(part 1 of 2)
# Autodesk Inventor assembly: Waffling60-MX
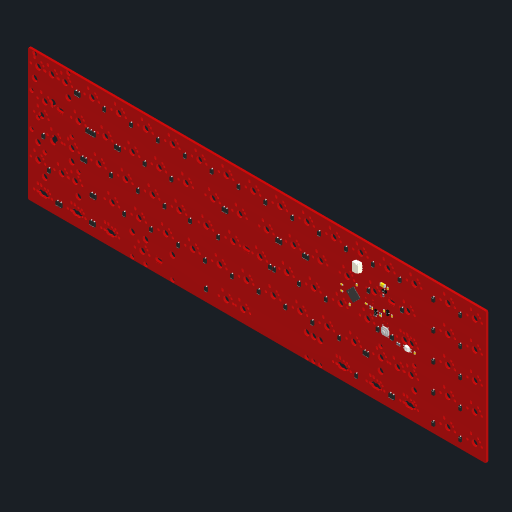
[picture p0: Inventor's stored thumbnail of the model, 512x512]
Saved by Autodesk Inventor 2024 (Build 280153000, 153)
## iProperties
Company: Open CASCADE
Created: 2024-04-27
Part Number: Waffling60-MX
Description: Open CASCADE Model
Document SubType Name: Assembly
Designer: bln15
Authority: Unknown
Sending System: Open CASCADE 7.5
Preprocessor: Open CASCADE STEP processor 7.5
Title: Open CASCADE Shape Model
Author: Author
## Documents named in this file (413)
- C:\Users\bln15\Documents\GitHub\waffling60\waffling60-XT\Waffling60-MX\Waffling60-MX.iam
- C:\Users\bln15\Documents\GitHub\waffling60\waffling60-XT\Waffling60-MX\Open CASCADE STEP translator 7.5 413.ipt
- C:\Users\bln15\Documents\GitHub\waffling60\waffling60-XT\Waffling60-MX\Open CASCADE STEP translator 7.5 414.ipt
- C:\Users\bln15\Documents\GitHub\waffling60\waffling60-XT\Waffling60-MX\Open CASCADE STEP translator 7.5 415.ipt
- C:\Users\bln15\Documents\GitHub\waffling60\waffling60-XT\Waffling60-MX\Open CASCADE STEP translator 7.5 416.ipt
- C:\Users\bln15\Documents\GitHub\waffling60\waffling60-XT\Waffling60-MX\Open CASCADE STEP translator 7.5 417.ipt
- C:\Users\bln15\Documents\GitHub\waffling60\waffling60-XT\Waffling60-MX\Open CASCADE STEP translator 7.5 418.ipt
- C:\Users\bln15\Documents\GitHub\waffling60\waffling60-XT\Waffling60-MX\Open CASCADE STEP translator 7.5 419.ipt
- C:\Users\bln15\Documents\GitHub\waffling60\waffling60-XT\Waffling60-MX\Open CASCADE STEP translator 7.5 420.ipt
- C:\Users\bln15\Documents\GitHub\waffling60\waffling60-XT\Waffling60-MX\Open CASCADE STEP translator 7.5 421.ipt
- C:\Users\bln15\Documents\GitHub\waffling60\waffling60-XT\Waffling60-MX\Open CASCADE STEP translator 7.5 422.ipt
- C:\Users\bln15\Documents\GitHub\waffling60\waffling60-XT\Waffling60-MX\Open CASCADE STEP translator 7.5 423.ipt
- C:\Users\bln15\Documents\GitHub\waffling60\waffling60-XT\Waffling60-MX\Open CASCADE STEP translator 7.5 424.ipt
- C:\Users\bln15\Documents\GitHub\waffling60\waffling60-XT\Waffling60-MX\Open CASCADE STEP translator 7.5 425.ipt
- C:\Users\bln15\Documents\GitHub\waffling60\waffling60-XT\Waffling60-MX\Open CASCADE STEP translator 7.5 426.ipt
- C:\Users\bln15\Documents\GitHub\waffling60\waffling60-XT\Waffling60-MX\Open CASCADE STEP translator 7.5 427.ipt
- C:\Users\bln15\Documents\GitHub\waffling60\waffling60-XT\Waffling60-MX\Open CASCADE STEP translator 7.5 428.ipt
- C:\Users\bln15\Documents\GitHub\waffling60\waffling60-XT\Waffling60-MX\Open CASCADE STEP translator 7.5 429.ipt
- C:\Users\bln15\Documents\GitHub\waffling60\waffling60-XT\Waffling60-MX\Open CASCADE STEP translator 7.5 430.ipt
- C:\Users\bln15\Documents\GitHub\waffling60\waffling60-XT\Waffling60-MX\Open CASCADE STEP translator 7.5 431.ipt
- C:\Users\bln15\Documents\GitHub\waffling60\waffling60-XT\Waffling60-MX\Open CASCADE STEP translator 7.5 432.ipt
- C:\Users\bln15\Documents\GitHub\waffling60\waffling60-XT\Waffling60-MX\Open CASCADE STEP translator 7.5 433.ipt
- C:\Users\bln15\Documents\GitHub\waffling60\waffling60-XT\Waffling60-MX\Open CASCADE STEP translator 7.5 434.ipt
- C:\Users\bln15\Documents\GitHub\waffling60\waffling60-XT\Waffling60-MX\Open CASCADE STEP translator 7.5 435.ipt
- C:\Users\bln15\Documents\GitHub\waffling60\waffling60-XT\Waffling60-MX\Open CASCADE STEP translator 7.5 436.ipt
- C:\Users\bln15\Documents\GitHub\waffling60\waffling60-XT\Waffling60-MX\Open CASCADE STEP translator 7.5 437.ipt
- C:\Users\bln15\Documents\GitHub\waffling60\waffling60-XT\Waffling60-MX\Open CASCADE STEP translator 7.5 438.ipt
- C:\Users\bln15\Documents\GitHub\waffling60\waffling60-XT\Waffling60-MX\Open CASCADE STEP translator 7.5 439.ipt
- C:\Users\bln15\Documents\GitHub\waffling60\waffling60-XT\Waffling60-MX\Open CASCADE STEP translator 7.5 440.ipt
- C:\Users\bln15\Documents\GitHub\waffling60\waffling60-XT\Waffling60-MX\Open CASCADE STEP translator 7.5 441.ipt
- C:\Users\bln15\Documents\GitHub\waffling60\waffling60-XT\Waffling60-MX\Open CASCADE STEP translator 7.5 442.ipt
- C:\Users\bln15\Documents\GitHub\waffling60\waffling60-XT\Waffling60-MX\Open CASCADE STEP translator 7.5 443.ipt
- C:\Users\bln15\Documents\GitHub\waffling60\waffling60-XT\Waffling60-MX\Open CASCADE STEP translator 7.5 444.ipt
- C:\Users\bln15\Documents\GitHub\waffling60\waffling60-XT\Waffling60-MX\Open CASCADE STEP translator 7.5 445.ipt
- C:\Users\bln15\Documents\GitHub\waffling60\waffling60-XT\Waffling60-MX\Open CASCADE STEP translator 7.5 446.ipt
- C:\Users\bln15\Documents\GitHub\waffling60\waffling60-XT\Waffling60-MX\Open CASCADE STEP translator 7.5 447.ipt
- C:\Users\bln15\Documents\GitHub\waffling60\waffling60-XT\Waffling60-MX\Open CASCADE STEP translator 7.5 448.ipt
- C:\Users\bln15\Documents\GitHub\waffling60\waffling60-XT\Waffling60-MX\Open CASCADE STEP translator 7.5 449.ipt
- C:\Users\bln15\Documents\GitHub\waffling60\waffling60-XT\Waffling60-MX\Open CASCADE STEP translator 7.5 450.ipt
- C:\Users\bln15\Documents\GitHub\waffling60\waffling60-XT\Waffling60-MX\Open CASCADE STEP translator 7.5 451.ipt
- C:\Users\bln15\Documents\GitHub\waffling60\waffling60-XT\Waffling60-MX\Open CASCADE STEP translator 7.5 452.ipt
- C:\Users\bln15\Documents\GitHub\waffling60\waffling60-XT\Waffling60-MX\Open CASCADE STEP translator 7.5 453.ipt
- C:\Users\bln15\Documents\GitHub\waffling60\waffling60-XT\Waffling60-MX\Open CASCADE STEP translator 7.5 454.ipt
- C:\Users\bln15\Documents\GitHub\waffling60\waffling60-XT\Waffling60-MX\Open CASCADE STEP translator 7.5 455.ipt
- C:\Users\bln15\Documents\GitHub\waffling60\waffling60-XT\Waffling60-MX\Open CASCADE STEP translator 7.5 456.ipt
- C:\Users\bln15\Documents\GitHub\waffling60\waffling60-XT\Waffling60-MX\Open CASCADE STEP translator 7.5 457.ipt
- C:\Users\bln15\Documents\GitHub\waffling60\waffling60-XT\Waffling60-MX\Open CASCADE STEP translator 7.5 458.ipt
- C:\Users\bln15\Documents\GitHub\waffling60\waffling60-XT\Waffling60-MX\Open CASCADE STEP translator 7.5 459.ipt
- C:\Users\bln15\Documents\GitHub\waffling60\waffling60-XT\Waffling60-MX\Open CASCADE STEP translator 7.5 460.ipt
- C:\Users\bln15\Documents\GitHub\waffling60\waffling60-XT\Waffling60-MX\Open CASCADE STEP translator 7.5 461.ipt
- C:\Users\bln15\Documents\GitHub\waffling60\waffling60-XT\Waffling60-MX\Open CASCADE STEP translator 7.5 462.ipt
- C:\Users\bln15\Documents\GitHub\waffling60\waffling60-XT\Waffling60-MX\Open CASCADE STEP translator 7.5 463.ipt
- C:\Users\bln15\Documents\GitHub\waffling60\waffling60-XT\Waffling60-MX\Open CASCADE STEP translator 7.5 464.ipt
- C:\Users\bln15\Documents\GitHub\waffling60\waffling60-XT\Waffling60-MX\Open CASCADE STEP translator 7.5 465.ipt
- C:\Users\bln15\Documents\GitHub\waffling60\waffling60-XT\Waffling60-MX\Open CASCADE STEP translator 7.5 466.ipt
- C:\Users\bln15\Documents\GitHub\waffling60\waffling60-XT\Waffling60-MX\Open CASCADE STEP translator 7.5 467.ipt
- C:\Users\bln15\Documents\GitHub\waffling60\waffling60-XT\Waffling60-MX\Open CASCADE STEP translator 7.5 468.ipt
- C:\Users\bln15\Documents\GitHub\waffling60\waffling60-XT\Waffling60-MX\Open CASCADE STEP translator 7.5 469.ipt
- C:\Users\bln15\Documents\GitHub\waffling60\waffling60-XT\Waffling60-MX\Open CASCADE STEP translator 7.5 470.ipt
- C:\Users\bln15\Documents\GitHub\waffling60\waffling60-XT\Waffling60-MX\Open CASCADE STEP translator 7.5 471.ipt
- C:\Users\bln15\Documents\GitHub\waffling60\waffling60-XT\Waffling60-MX\Open CASCADE STEP translator 7.5 472.ipt
- C:\Users\bln15\Documents\GitHub\waffling60\waffling60-XT\Waffling60-MX\Open CASCADE STEP translator 7.5 473.ipt
- C:\Users\bln15\Documents\GitHub\waffling60\waffling60-XT\Waffling60-MX\Open CASCADE STEP translator 7.5 474.ipt
- C:\Users\bln15\Documents\GitHub\waffling60\waffling60-XT\Waffling60-MX\Open CASCADE STEP translator 7.5 475.ipt
- C:\Users\bln15\Documents\GitHub\waffling60\waffling60-XT\Waffling60-MX\Open CASCADE STEP translator 7.5 476.ipt
- C:\Users\bln15\Documents\GitHub\waffling60\waffling60-XT\Waffling60-MX\Open CASCADE STEP translator 7.5 477.ipt
- C:\Users\bln15\Documents\GitHub\waffling60\waffling60-XT\Waffling60-MX\Open CASCADE STEP translator 7.5 478.ipt
- C:\Users\bln15\Documents\GitHub\waffling60\waffling60-XT\Waffling60-MX\Open CASCADE STEP translator 7.5 479.ipt
- C:\Users\bln15\Documents\GitHub\waffling60\waffling60-XT\Waffling60-MX\Open CASCADE STEP translator 7.5 480.ipt
- C:\Users\bln15\Documents\GitHub\waffling60\waffling60-XT\Waffling60-MX\Open CASCADE STEP translator 7.5 481.ipt
- C:\Users\bln15\Documents\GitHub\waffling60\waffling60-XT\Waffling60-MX\Open CASCADE STEP translator 7.5 482.ipt
- C:\Users\bln15\Documents\GitHub\waffling60\waffling60-XT\Waffling60-MX\Open CASCADE STEP translator 7.5 483.ipt
- C:\Users\bln15\Documents\GitHub\waffling60\waffling60-XT\Waffling60-MX\Open CASCADE STEP translator 7.5 484.ipt
- C:\Users\bln15\Documents\GitHub\waffling60\waffling60-XT\Waffling60-MX\Open CASCADE STEP translator 7.5 485.ipt
- C:\Users\bln15\Documents\GitHub\waffling60\waffling60-XT\Waffling60-MX\Open CASCADE STEP translator 7.5 486.ipt
- C:\Users\bln15\Documents\GitHub\waffling60\waffling60-XT\Waffling60-MX\Open CASCADE STEP translator 7.5 487.ipt
- C:\Users\bln15\Documents\GitHub\waffling60\waffling60-XT\Waffling60-MX\Open CASCADE STEP translator 7.5 488.ipt
- C:\Users\bln15\Documents\GitHub\waffling60\waffling60-XT\Waffling60-MX\Open CASCADE STEP translator 7.5 489.ipt
- C:\Users\bln15\Documents\GitHub\waffling60\waffling60-XT\Waffling60-MX\Open CASCADE STEP translator 7.5 490.ipt
- C:\Users\bln15\Documents\GitHub\waffling60\waffling60-XT\Waffling60-MX\Open CASCADE STEP translator 7.5 491.ipt
- C:\Users\bln15\Documents\GitHub\waffling60\waffling60-XT\Waffling60-MX\Open CASCADE STEP translator 7.5 492.ipt
- C:\Users\bln15\Documents\GitHub\waffling60\waffling60-XT\Waffling60-MX\Open CASCADE STEP translator 7.5 493.ipt
- C:\Users\bln15\Documents\GitHub\waffling60\waffling60-XT\Waffling60-MX\Open CASCADE STEP translator 7.5 494.ipt
- C:\Users\bln15\Documents\GitHub\waffling60\waffling60-XT\Waffling60-MX\Open CASCADE STEP translator 7.5 495.ipt
- C:\Users\bln15\Documents\GitHub\waffling60\waffling60-XT\Waffling60-MX\Open CASCADE STEP translator 7.5 496.ipt
- C:\Users\bln15\Documents\GitHub\waffling60\waffling60-XT\Waffling60-MX\Open CASCADE STEP translator 7.5 497.ipt
- C:\Users\bln15\Documents\GitHub\waffling60\waffling60-XT\Waffling60-MX\Open CASCADE STEP translator 7.5 498.ipt
- C:\Users\bln15\Documents\GitHub\waffling60\waffling60-XT\Waffling60-MX\Open CASCADE STEP translator 7.5 499.ipt
- C:\Users\bln15\Documents\GitHub\waffling60\waffling60-XT\Waffling60-MX\Open CASCADE STEP translator 7.5 500.ipt
- C:\Users\bln15\Documents\GitHub\waffling60\waffling60-XT\Waffling60-MX\Open CASCADE STEP translator 7.5 501.ipt
- C:\Users\bln15\Documents\GitHub\waffling60\waffling60-XT\Waffling60-MX\Open CASCADE STEP translator 7.5 502.ipt
- C:\Users\bln15\Documents\GitHub\waffling60\waffling60-XT\Waffling60-MX\Open CASCADE STEP translator 7.5 503.ipt
- C:\Users\bln15\Documents\GitHub\waffling60\waffling60-XT\Waffling60-MX\Open CASCADE STEP translator 7.5 504.ipt
- C:\Users\bln15\Documents\GitHub\waffling60\waffling60-XT\Waffling60-MX\Open CASCADE STEP translator 7.5 505.ipt
- C:\Users\bln15\Documents\GitHub\waffling60\waffling60-XT\Waffling60-MX\Open CASCADE STEP translator 7.5 506.ipt
- C:\Users\bln15\Documents\GitHub\waffling60\waffling60-XT\Waffling60-MX\Open CASCADE STEP translator 7.5 507.ipt
- C:\Users\bln15\Documents\GitHub\waffling60\waffling60-XT\Waffling60-MX\Open CASCADE STEP translator 7.5 508.ipt
- C:\Users\bln15\Documents\GitHub\waffling60\waffling60-XT\Waffling60-MX\Open CASCADE STEP translator 7.5 509.ipt
- C:\Users\bln15\Documents\GitHub\waffling60\waffling60-XT\Waffling60-MX\Open CASCADE STEP translator 7.5 510.ipt
- C:\Users\bln15\Documents\GitHub\waffling60\waffling60-XT\Waffling60-MX\Open CASCADE STEP translator 7.5 511.ipt
- C:\Users\bln15\Documents\GitHub\waffling60\waffling60-XT\Waffling60-MX\Open CASCADE STEP translator 7.5 512.ipt
- C:\Users\bln15\Documents\GitHub\waffling60\waffling60-XT\Waffling60-MX\Open CASCADE STEP translator 7.5 513.ipt
- C:\Users\bln15\Documents\GitHub\waffling60\waffling60-XT\Waffling60-MX\Open CASCADE STEP translator 7.5 514.ipt
- C:\Users\bln15\Documents\GitHub\waffling60\waffling60-XT\Waffling60-MX\Open CASCADE STEP translator 7.5 515.ipt
- C:\Users\bln15\Documents\GitHub\waffling60\waffling60-XT\Waffling60-MX\Open CASCADE STEP translator 7.5 516.ipt
- C:\Users\bln15\Documents\GitHub\waffling60\waffling60-XT\Waffling60-MX\Open CASCADE STEP translator 7.5 517.ipt
- C:\Users\bln15\Documents\GitHub\waffling60\waffling60-XT\Waffling60-MX\Open CASCADE STEP translator 7.5 518.ipt
- C:\Users\bln15\Documents\GitHub\waffling60\waffling60-XT\Waffling60-MX\Open CASCADE STEP translator 7.5 519.ipt
- C:\Users\bln15\Documents\GitHub\waffling60\waffling60-XT\Waffling60-MX\Open CASCADE STEP translator 7.5 520.ipt
- C:\Users\bln15\Documents\GitHub\waffling60\waffling60-XT\Waffling60-MX\Open CASCADE STEP translator 7.5 521.ipt
- C:\Users\bln15\Documents\GitHub\waffling60\waffling60-XT\Waffling60-MX\Open CASCADE STEP translator 7.5 522.ipt
- C:\Users\bln15\Documents\GitHub\waffling60\waffling60-XT\Waffling60-MX\Open CASCADE STEP translator 7.5 523.ipt
- C:\Users\bln15\Documents\GitHub\waffling60\waffling60-XT\Waffling60-MX\Open CASCADE STEP translator 7.5 524.ipt
- C:\Users\bln15\Documents\GitHub\waffling60\waffling60-XT\Waffling60-MX\Open CASCADE STEP translator 7.5 525.ipt
- C:\Users\bln15\Documents\GitHub\waffling60\waffling60-XT\Waffling60-MX\Open CASCADE STEP translator 7.5 526.ipt
- C:\Users\bln15\Documents\GitHub\waffling60\waffling60-XT\Waffling60-MX\Open CASCADE STEP translator 7.5 527.ipt
- C:\Users\bln15\Documents\GitHub\waffling60\waffling60-XT\Waffling60-MX\Open CASCADE STEP translator 7.5 528.ipt
- C:\Users\bln15\Documents\GitHub\waffling60\waffling60-XT\Waffling60-MX\Open CASCADE STEP translator 7.5 529.ipt
- C:\Users\bln15\Documents\GitHub\waffling60\waffling60-XT\Waffling60-MX\Open CASCADE STEP translator 7.5 530.ipt
- C:\Users\bln15\Documents\GitHub\waffling60\waffling60-XT\Waffling60-MX\Open CASCADE STEP translator 7.5 531.ipt
- C:\Users\bln15\Documents\GitHub\waffling60\waffling60-XT\Waffling60-MX\Open CASCADE STEP translator 7.5 532.ipt
- C:\Users\bln15\Documents\GitHub\waffling60\waffling60-XT\Waffling60-MX\Open CASCADE STEP translator 7.5 533.ipt
- C:\Users\bln15\Documents\GitHub\waffling60\waffling60-XT\Waffling60-MX\Open CASCADE STEP translator 7.5 534.ipt
- C:\Users\bln15\Documents\GitHub\waffling60\waffling60-XT\Waffling60-MX\Open CASCADE STEP translator 7.5 535.ipt
- C:\Users\bln15\Documents\GitHub\waffling60\waffling60-XT\Waffling60-MX\Open CASCADE STEP translator 7.5 536.ipt
- C:\Users\bln15\Documents\GitHub\waffling60\waffling60-XT\Waffling60-MX\Open CASCADE STEP translator 7.5 537.ipt
- C:\Users\bln15\Documents\GitHub\waffling60\waffling60-XT\Waffling60-MX\Open CASCADE STEP translator 7.5 538.ipt
- C:\Users\bln15\Documents\GitHub\waffling60\waffling60-XT\Waffling60-MX\Open CASCADE STEP translator 7.5 539.ipt
- C:\Users\bln15\Documents\GitHub\waffling60\waffling60-XT\Waffling60-MX\Open CASCADE STEP translator 7.5 540.ipt
- C:\Users\bln15\Documents\GitHub\waffling60\waffling60-XT\Waffling60-MX\Open CASCADE STEP translator 7.5 541.ipt
- C:\Users\bln15\Documents\GitHub\waffling60\waffling60-XT\Waffling60-MX\Open CASCADE STEP translator 7.5 542.ipt
- C:\Users\bln15\Documents\GitHub\waffling60\waffling60-XT\Waffling60-MX\Open CASCADE STEP translator 7.5 543.ipt
- C:\Users\bln15\Documents\GitHub\waffling60\waffling60-XT\Waffling60-MX\Open CASCADE STEP translator 7.5 544.ipt
- C:\Users\bln15\Documents\GitHub\waffling60\waffling60-XT\Waffling60-MX\Open CASCADE STEP translator 7.5 545.ipt
- C:\Users\bln15\Documents\GitHub\waffling60\waffling60-XT\Waffling60-MX\Open CASCADE STEP translator 7.5 546.ipt
- C:\Users\bln15\Documents\GitHub\waffling60\waffling60-XT\Waffling60-MX\Open CASCADE STEP translator 7.5 547.ipt
- C:\Users\bln15\Documents\GitHub\waffling60\waffling60-XT\Waffling60-MX\Open CASCADE STEP translator 7.5 548.ipt
- C:\Users\bln15\Documents\GitHub\waffling60\waffling60-XT\Waffling60-MX\Open CASCADE STEP translator 7.5 549.ipt
- C:\Users\bln15\Documents\GitHub\waffling60\waffling60-XT\Waffling60-MX\Open CASCADE STEP translator 7.5 550.ipt
- C:\Users\bln15\Documents\GitHub\waffling60\waffling60-XT\Waffling60-MX\Open CASCADE STEP translator 7.5 551.ipt
- C:\Users\bln15\Documents\GitHub\waffling60\waffling60-XT\Waffling60-MX\Open CASCADE STEP translator 7.5 552.ipt
- C:\Users\bln15\Documents\GitHub\waffling60\waffling60-XT\Waffling60-MX\Open CASCADE STEP translator 7.5 553.ipt
- C:\Users\bln15\Documents\GitHub\waffling60\waffling60-XT\Waffling60-MX\Open CASCADE STEP translator 7.5 554.ipt
- C:\Users\bln15\Documents\GitHub\waffling60\waffling60-XT\Waffling60-MX\Open CASCADE STEP translator 7.5 555.ipt
- C:\Users\bln15\Documents\GitHub\waffling60\waffling60-XT\Waffling60-MX\Open CASCADE STEP translator 7.5 556.ipt
- C:\Users\bln15\Documents\GitHub\waffling60\waffling60-XT\Waffling60-MX\Open CASCADE STEP translator 7.5 557.ipt
- C:\Users\bln15\Documents\GitHub\waffling60\waffling60-XT\Waffling60-MX\Open CASCADE STEP translator 7.5 558.ipt
- C:\Users\bln15\Documents\GitHub\waffling60\waffling60-XT\Waffling60-MX\Open CASCADE STEP translator 7.5 559.ipt
- C:\Users\bln15\Documents\GitHub\waffling60\waffling60-XT\Waffling60-MX\Open CASCADE STEP translator 7.5 560.ipt
- C:\Users\bln15\Documents\GitHub\waffling60\waffling60-XT\Waffling60-MX\Open CASCADE STEP translator 7.5 561.ipt
- C:\Users\bln15\Documents\GitHub\waffling60\waffling60-XT\Waffling60-MX\Open CASCADE STEP translator 7.5 562.ipt
- C:\Users\bln15\Documents\GitHub\waffling60\waffling60-XT\Waffling60-MX\Open CASCADE STEP translator 7.5 563.ipt
- C:\Users\bln15\Documents\GitHub\waffling60\waffling60-XT\Waffling60-MX\Open CASCADE STEP translator 7.5 564.ipt
- C:\Users\bln15\Documents\GitHub\waffling60\waffling60-XT\Waffling60-MX\Open CASCADE STEP translator 7.5 565.ipt
- C:\Users\bln15\Documents\GitHub\waffling60\waffling60-XT\Waffling60-MX\Open CASCADE STEP translator 7.5 566.ipt
- C:\Users\bln15\Documents\GitHub\waffling60\waffling60-XT\Waffling60-MX\Open CASCADE STEP translator 7.5 567.ipt
- C:\Users\bln15\Documents\GitHub\waffling60\waffling60-XT\Waffling60-MX\Open CASCADE STEP translator 7.5 568.ipt
- C:\Users\bln15\Documents\GitHub\waffling60\waffling60-XT\Waffling60-MX\Open CASCADE STEP translator 7.5 569.ipt
- C:\Users\bln15\Documents\GitHub\waffling60\waffling60-XT\Waffling60-MX\Open CASCADE STEP translator 7.5 570.ipt
- C:\Users\bln15\Documents\GitHub\waffling60\waffling60-XT\Waffling60-MX\Open CASCADE STEP translator 7.5 571.ipt
- C:\Users\bln15\Documents\GitHub\waffling60\waffling60-XT\Waffling60-MX\Open CASCADE STEP translator 7.5 572.ipt
- C:\Users\bln15\Documents\GitHub\waffling60\waffling60-XT\Waffling60-MX\Open CASCADE STEP translator 7.5 573.ipt
- C:\Users\bln15\Documents\GitHub\waffling60\waffling60-XT\Waffling60-MX\Open CASCADE STEP translator 7.5 574.ipt
- C:\Users\bln15\Documents\GitHub\waffling60\waffling60-XT\Waffling60-MX\Open CASCADE STEP translator 7.5 575.ipt
- C:\Users\bln15\Documents\GitHub\waffling60\waffling60-XT\Waffling60-MX\Open CASCADE STEP translator 7.5 576.ipt
- C:\Users\bln15\Documents\GitHub\waffling60\waffling60-XT\Waffling60-MX\Open CASCADE STEP translator 7.5 577.ipt
- C:\Users\bln15\Documents\GitHub\waffling60\waffling60-XT\Waffling60-MX\Open CASCADE STEP translator 7.5 578.ipt
- C:\Users\bln15\Documents\GitHub\waffling60\waffling60-XT\Waffling60-MX\Open CASCADE STEP translator 7.5 579.ipt
- C:\Users\bln15\Documents\GitHub\waffling60\waffling60-XT\Waffling60-MX\Open CASCADE STEP translator 7.5 580.ipt
- C:\Users\bln15\Documents\GitHub\waffling60\waffling60-XT\Waffling60-MX\Open CASCADE STEP translator 7.5 581.ipt
- C:\Users\bln15\Documents\GitHub\waffling60\waffling60-XT\Waffling60-MX\Open CASCADE STEP translator 7.5 582.ipt
- C:\Users\bln15\Documents\GitHub\waffling60\waffling60-XT\Waffling60-MX\Open CASCADE STEP translator 7.5 583.ipt
- C:\Users\bln15\Documents\GitHub\waffling60\waffling60-XT\Waffling60-MX\Open CASCADE STEP translator 7.5 584.ipt
- C:\Users\bln15\Documents\GitHub\waffling60\waffling60-XT\Waffling60-MX\Open CASCADE STEP translator 7.5 585.ipt
- C:\Users\bln15\Documents\GitHub\waffling60\waffling60-XT\Waffling60-MX\Open CASCADE STEP translator 7.5 586.ipt
- C:\Users\bln15\Documents\GitHub\waffling60\waffling60-XT\Waffling60-MX\Open CASCADE STEP translator 7.5 587.ipt
- C:\Users\bln15\Documents\GitHub\waffling60\waffling60-XT\Waffling60-MX\Open CASCADE STEP translator 7.5 588.ipt
- C:\Users\bln15\Documents\GitHub\waffling60\waffling60-XT\Waffling60-MX\Open CASCADE STEP translator 7.5 589.ipt
- C:\Users\bln15\Documents\GitHub\waffling60\waffling60-XT\Waffling60-MX\Open CASCADE STEP translator 7.5 590.ipt
- C:\Users\bln15\Documents\GitHub\waffling60\waffling60-XT\Waffling60-MX\Open CASCADE STEP translator 7.5 591.ipt
- C:\Users\bln15\Documents\GitHub\waffling60\waffling60-XT\Waffling60-MX\Open CASCADE STEP translator 7.5 592.ipt
- C:\Users\bln15\Documents\GitHub\waffling60\waffling60-XT\Waffling60-MX\Open CASCADE STEP translator 7.5 593.ipt
- C:\Users\bln15\Documents\GitHub\waffling60\waffling60-XT\Waffling60-MX\Open CASCADE STEP translator 7.5 594.ipt
- C:\Users\bln15\Documents\GitHub\waffling60\waffling60-XT\Waffling60-MX\Open CASCADE STEP translator 7.5 595.ipt
- C:\Users\bln15\Documents\GitHub\waffling60\waffling60-XT\Waffling60-MX\Open CASCADE STEP translator 7.5 596.ipt
- C:\Users\bln15\Documents\GitHub\waffling60\waffling60-XT\Waffling60-MX\Open CASCADE STEP translator 7.5 597.ipt
- C:\Users\bln15\Documents\GitHub\waffling60\waffling60-XT\Waffling60-MX\Open CASCADE STEP translator 7.5 598.ipt
- C:\Users\bln15\Documents\GitHub\waffling60\waffling60-XT\Waffling60-MX\Open CASCADE STEP translator 7.5 599.ipt
- C:\Users\bln15\Documents\GitHub\waffling60\waffling60-XT\Waffling60-MX\Open CASCADE STEP translator 7.5 600.ipt
- C:\Users\bln15\Documents\GitHub\waffling60\waffling60-XT\Waffling60-MX\Open CASCADE STEP translator 7.5 601.ipt
- C:\Users\bln15\Documents\GitHub\waffling60\waffling60-XT\Waffling60-MX\Open CASCADE STEP translator 7.5 602.ipt
- C:\Users\bln15\Documents\GitHub\waffling60\waffling60-XT\Waffling60-MX\Open CASCADE STEP translator 7.5 603.ipt
- C:\Users\bln15\Documents\GitHub\waffling60\waffling60-XT\Waffling60-MX\Open CASCADE STEP translator 7.5 604.ipt
- C:\Users\bln15\Documents\GitHub\waffling60\waffling60-XT\Waffling60-MX\Open CASCADE STEP translator 7.5 605.ipt
- C:\Users\bln15\Documents\GitHub\waffling60\waffling60-XT\Waffling60-MX\Open CASCADE STEP translator 7.5 606.ipt
- C:\Users\bln15\Documents\GitHub\waffling60\waffling60-XT\Waffling60-MX\Open CASCADE STEP translator 7.5 607.ipt
- C:\Users\bln15\Documents\GitHub\waffling60\waffling60-XT\Waffling60-MX\Open CASCADE STEP translator 7.5 608.ipt
- C:\Users\bln15\Documents\GitHub\waffling60\waffling60-XT\Waffling60-MX\Open CASCADE STEP translator 7.5 609.ipt
- C:\Users\bln15\Documents\GitHub\waffling60\waffling60-XT\Waffling60-MX\Open CASCADE STEP translator 7.5 610.ipt
- C:\Users\bln15\Documents\GitHub\waffling60\waffling60-XT\Waffling60-MX\Open CASCADE STEP translator 7.5 611.ipt
- C:\Users\bln15\Documents\GitHub\waffling60\waffling60-XT\Waffling60-MX\Open CASCADE STEP translator 7.5 612.ipt
- C:\Users\bln15\Documents\GitHub\waffling60\waffling60-XT\Waffling60-MX\Open CASCADE STEP translator 7.5 613.ipt
- C:\Users\bln15\Documents\GitHub\waffling60\waffling60-XT\Waffling60-MX\Open CASCADE STEP translator 7.5 614.ipt
- C:\Users\bln15\Documents\GitHub\waffling60\waffling60-XT\Waffling60-MX\Open CASCADE STEP translator 7.5 615.ipt
- C:\Users\bln15\Documents\GitHub\waffling60\waffling60-XT\Waffling60-MX\Open CASCADE STEP translator 7.5 616.ipt
- C:\Users\bln15\Documents\GitHub\waffling60\waffling60-XT\Waffling60-MX\Open CASCADE STEP translator 7.5 617.ipt
- C:\Users\bln15\Documents\GitHub\waffling60\waffling60-XT\Waffling60-MX\Open CASCADE STEP translator 7.5 618.ipt
- C:\Users\bln15\Documents\GitHub\waffling60\waffling60-XT\Waffling60-MX\Open CASCADE STEP translator 7.5 619.ipt
- C:\Users\bln15\Documents\GitHub\waffling60\waffling60-XT\Waffling60-MX\Open CASCADE STEP translator 7.5 620.ipt
- C:\Users\bln15\Documents\GitHub\waffling60\waffling60-XT\Waffling60-MX\Open CASCADE STEP translator 7.5 621.ipt
- C:\Users\bln15\Documents\GitHub\waffling60\waffling60-XT\Waffling60-MX\Open CASCADE STEP translator 7.5 622.ipt
- C:\Users\bln15\Documents\GitHub\waffling60\waffling60-XT\Waffling60-MX\Open CASCADE STEP translator 7.5 623.ipt
- C:\Users\bln15\Documents\GitHub\waffling60\waffling60-XT\Waffling60-MX\Open CASCADE STEP translator 7.5 624.ipt
- C:\Users\bln15\Documents\GitHub\waffling60\waffling60-XT\Waffling60-MX\Open CASCADE STEP translator 7.5 625.ipt
- C:\Users\bln15\Documents\GitHub\waffling60\waffling60-XT\Waffling60-MX\Open CASCADE STEP translator 7.5 626.ipt
- C:\Users\bln15\Documents\GitHub\waffling60\waffling60-XT\Waffling60-MX\Open CASCADE STEP translator 7.5 627.ipt
- C:\Users\bln15\Documents\GitHub\waffling60\waffling60-XT\Waffling60-MX\Open CASCADE STEP translator 7.5 628.ipt
- C:\Users\bln15\Documents\GitHub\waffling60\waffling60-XT\Waffling60-MX\Open CASCADE STEP translator 7.5 629.ipt
- C:\Users\bln15\Documents\GitHub\waffling60\waffling60-XT\Waffling60-MX\Open CASCADE STEP translator 7.5 630.ipt
- C:\Users\bln15\Documents\GitHub\waffling60\waffling60-XT\Waffling60-MX\Open CASCADE STEP translator 7.5 631.ipt
- C:\Users\bln15\Documents\GitHub\waffling60\waffling60-XT\Waffling60-MX\Open CASCADE STEP translator 7.5 632.ipt
- C:\Users\bln15\Documents\GitHub\waffling60\waffling60-XT\Waffling60-MX\Open CASCADE STEP translator 7.5 633.ipt
- C:\Users\bln15\Documents\GitHub\waffling60\waffling60-XT\Waffling60-MX\Open CASCADE STEP translator 7.5 634.ipt
- C:\Users\bln15\Documents\GitHub\waffling60\waffling60-XT\Waffling60-MX\Open CASCADE STEP translator 7.5 635.ipt
- C:\Users\bln15\Documents\GitHub\waffling60\waffling60-XT\Waffling60-MX\Open CASCADE STEP translator 7.5 636.ipt
- C:\Users\bln15\Documents\GitHub\waffling60\waffling60-XT\Waffling60-MX\Open CASCADE STEP translator 7.5 637.ipt
- C:\Users\bln15\Documents\GitHub\waffling60\waffling60-XT\Waffling60-MX\Open CASCADE STEP translator 7.5 638.ipt
- C:\Users\bln15\Documents\GitHub\waffling60\waffling60-XT\Waffling60-MX\Open CASCADE STEP translator 7.5 639.ipt
- C:\Users\bln15\Documents\GitHub\waffling60\waffling60-XT\Waffling60-MX\Open CASCADE STEP translator 7.5 640.ipt
- C:\Users\bln15\Documents\GitHub\waffling60\waffling60-XT\Waffling60-MX\Open CASCADE STEP translator 7.5 641.ipt
- C:\Users\bln15\Documents\GitHub\waffling60\waffling60-XT\Waffling60-MX\Open CASCADE STEP translator 7.5 642.ipt
- C:\Users\bln15\Documents\GitHub\waffling60\waffling60-XT\Waffling60-MX\Open CASCADE STEP translator 7.5 643.ipt
- C:\Users\bln15\Documents\GitHub\waffling60\waffling60-XT\Waffling60-MX\Open CASCADE STEP translator 7.5 644.ipt
- C:\Users\bln15\Documents\GitHub\waffling60\waffling60-XT\Waffling60-MX\Open CASCADE STEP translator 7.5 645.ipt
- C:\Users\bln15\Documents\GitHub\waffling60\waffling60-XT\Waffling60-MX\Open CASCADE STEP translator 7.5 646.ipt
- C:\Users\bln15\Documents\GitHub\waffling60\waffling60-XT\Waffling60-MX\Open CASCADE STEP translator 7.5 647.ipt
- C:\Users\bln15\Documents\GitHub\waffling60\waffling60-XT\Waffling60-MX\Open CASCADE STEP translator 7.5 648.ipt
- C:\Users\bln15\Documents\GitHub\waffling60\waffling60-XT\Waffling60-MX\Open CASCADE STEP translator 7.5 649.ipt
- C:\Users\bln15\Documents\GitHub\waffling60\waffling60-XT\Waffling60-MX\Open CASCADE STEP translator 7.5 650.ipt
- C:\Users\bln15\Documents\GitHub\waffling60\waffling60-XT\Waffling60-MX\Open CASCADE STEP translator 7.5 651.ipt
- C:\Users\bln15\Documents\GitHub\waffling60\waffling60-XT\Waffling60-MX\Open CASCADE STEP translator 7.5 652.ipt
- C:\Users\bln15\Documents\GitHub\waffling60\waffling60-XT\Waffling60-MX\Open CASCADE STEP translator 7.5 653.ipt
- C:\Users\bln15\Documents\GitHub\waffling60\waffling60-XT\Waffling60-MX\Open CASCADE STEP translator 7.5 654.ipt
- C:\Users\bln15\Documents\GitHub\waffling60\waffling60-XT\Waffling60-MX\Open CASCADE STEP translator 7.5 655.ipt
- C:\Users\bln15\Documents\GitHub\waffling60\waffling60-XT\Waffling60-MX\Open CASCADE STEP translator 7.5 656.ipt
- C:\Users\bln15\Documents\GitHub\waffling60\waffling60-XT\Waffling60-MX\Open CASCADE STEP translator 7.5 657.ipt
- C:\Users\bln15\Documents\GitHub\waffling60\waffling60-XT\Waffling60-MX\Open CASCADE STEP translator 7.5 658.ipt
- C:\Users\bln15\Documents\GitHub\waffling60\waffling60-XT\Waffling60-MX\Open CASCADE STEP translator 7.5 659.ipt
- C:\Users\bln15\Documents\GitHub\waffling60\waffling60-XT\Waffling60-MX\Open CASCADE STEP translator 7.5 660.ipt
- C:\Users\bln15\Documents\GitHub\waffling60\waffling60-XT\Waffling60-MX\Open CASCADE STEP translator 7.5 661.ipt
- C:\Users\bln15\Documents\GitHub\waffling60\waffling60-XT\Waffling60-MX\Open CASCADE STEP translator 7.5 662.ipt
- C:\Users\bln15\Documents\GitHub\waffling60\waffling60-XT\Waffling60-MX\Open CASCADE STEP translator 7.5 663.ipt
- C:\Users\bln15\Documents\GitHub\waffling60\waffling60-XT\Waffling60-MX\Open CASCADE STEP translator 7.5 664.ipt
- C:\Users\bln15\Documents\GitHub\waffling60\waffling60-XT\Waffling60-MX\Open CASCADE STEP translator 7.5 665.ipt
- C:\Users\bln15\Documents\GitHub\waffling60\waffling60-XT\Waffling60-MX\Open CASCADE STEP translator 7.5 666.ipt
- C:\Users\bln15\Documents\GitHub\waffling60\waffling60-XT\Waffling60-MX\Open CASCADE STEP translator 7.5 667.ipt
- C:\Users\bln15\Documents\GitHub\waffling60\waffling60-XT\Waffling60-MX\Open CASCADE STEP translator 7.5 668.ipt
- C:\Users\bln15\Documents\GitHub\waffling60\waffling60-XT\Waffling60-MX\Open CASCADE STEP translator 7.5 669.ipt
- C:\Users\bln15\Documents\GitHub\waffling60\waffling60-XT\Waffling60-MX\Open CASCADE STEP translator 7.5 670.ipt
- C:\Users\bln15\Documents\GitHub\waffling60\waffling60-XT\Waffling60-MX\Open CASCADE STEP translator 7.5 671.ipt
- C:\Users\bln15\Documents\GitHub\waffling60\waffling60-XT\Waffling60-MX\Open CASCADE STEP translator 7.5 672.ipt
- C:\Users\bln15\Documents\GitHub\waffling60\waffling60-XT\Waffling60-MX\Open CASCADE STEP translator 7.5 673.ipt
- C:\Users\bln15\Documents\GitHub\waffling60\waffling60-XT\Waffling60-MX\Open CASCADE STEP translator 7.5 674.ipt
- C:\Users\bln15\Documents\GitHub\waffling60\waffling60-XT\Waffling60-MX\Open CASCADE STEP translator 7.5 675.ipt
- C:\Users\bln15\Documents\GitHub\waffling60\waffling60-XT\Waffling60-MX\Open CASCADE STEP translator 7.5 676.ipt
- C:\Users\bln15\Documents\GitHub\waffling60\waffling60-XT\Waffling60-MX\Open CASCADE STEP translator 7.5 677.ipt
- C:\Users\bln15\Documents\GitHub\waffling60\waffling60-XT\Waffling60-MX\Open CASCADE STEP translator 7.5 678.ipt
- C:\Users\bln15\Documents\GitHub\waffling60\waffling60-XT\Waffling60-MX\Open CASCADE STEP translator 7.5 679.ipt
- C:\Users\bln15\Documents\GitHub\waffling60\waffling60-XT\Waffling60-MX\Open CASCADE STEP translator 7.5 680.ipt
- C:\Users\bln15\Documents\GitHub\waffling60\waffling60-XT\Waffling60-MX\Open CASCADE STEP translator 7.5 681.ipt
- C:\Users\bln15\Documents\GitHub\waffling60\waffling60-XT\Waffling60-MX\Open CASCADE STEP translator 7.5 682.ipt
- C:\Users\bln15\Documents\GitHub\waffling60\waffling60-XT\Waffling60-MX\Open CASCADE STEP translator 7.5 683.ipt
- C:\Users\bln15\Documents\GitHub\waffling60\waffling60-XT\Waffling60-MX\Open CASCADE STEP translator 7.5 684.ipt
- C:\Users\bln15\Documents\GitHub\waffling60\waffling60-XT\Waffling60-MX\Open CASCADE STEP translator 7.5 685.ipt
- C:\Users\bln15\Documents\GitHub\waffling60\waffling60-XT\Waffling60-MX\Open CASCADE STEP translator 7.5 686.ipt
- C:\Users\bln15\Documents\GitHub\waffling60\waffling60-XT\Waffling60-MX\Open CASCADE STEP translator 7.5 687.ipt
- C:\Users\bln15\Documents\GitHub\waffling60\waffling60-XT\Waffling60-MX\Open CASCADE STEP translator 7.5 688.ipt
- C:\Users\bln15\Documents\GitHub\waffling60\waffling60-XT\Waffling60-MX\Open CASCADE STEP translator 7.5 689.ipt
- C:\Users\bln15\Documents\GitHub\waffling60\waffling60-XT\Waffling60-MX\Open CASCADE STEP translator 7.5 690.ipt
- C:\Users\bln15\Documents\GitHub\waffling60\waffling60-XT\Waffling60-MX\Open CASCADE STEP translator 7.5 691.ipt
- C:\Users\bln15\Documents\GitHub\waffling60\waffling60-XT\Waffling60-MX\Open CASCADE STEP translator 7.5 692.ipt
- C:\Users\bln15\Documents\GitHub\waffling60\waffling60-XT\Waffling60-MX\Open CASCADE STEP translator 7.5 693.ipt
- C:\Users\bln15\Documents\GitHub\waffling60\waffling60-XT\Waffling60-MX\Open CASCADE STEP translator 7.5 694.ipt
- C:\Users\bln15\Documents\GitHub\waffling60\waffling60-XT\Waffling60-MX\Open CASCADE STEP translator 7.5 695.ipt
- C:\Users\bln15\Documents\GitHub\waffling60\waffling60-XT\Waffling60-MX\Open CASCADE STEP translator 7.5 696.ipt
- C:\Users\bln15\Documents\GitHub\waffling60\waffling60-XT\Waffling60-MX\Open CASCADE STEP translator 7.5 697.ipt
- C:\Users\bln15\Documents\GitHub\waffling60\waffling60-XT\Waffling60-MX\Open CASCADE STEP translator 7.5 698.ipt
- C:\Users\bln15\Documents\GitHub\waffling60\waffling60-XT\Waffling60-MX\Open CASCADE STEP translator 7.5 699.ipt
- C:\Users\bln15\Documents\GitHub\waffling60\waffling60-XT\Waffling60-MX\Open CASCADE STEP translator 7.5 700.ipt
- C:\Users\bln15\Documents\GitHub\waffling60\waffling60-XT\Waffling60-MX\Open CASCADE STEP translator 7.5 701.ipt
- C:\Users\bln15\Documents\GitHub\waffling60\waffling60-XT\Waffling60-MX\Open CASCADE STEP translator 7.5 702.ipt
- C:\Users\bln15\Documents\GitHub\waffling60\waffling60-XT\Waffling60-MX\Open CASCADE STEP translator 7.5 703.ipt
- C:\Users\bln15\Documents\GitHub\waffling60\waffling60-XT\Waffling60-MX\Open CASCADE STEP translator 7.5 704.ipt
- C:\Users\bln15\Documents\GitHub\waffling60\waffling60-XT\Waffling60-MX\Open CASCADE STEP translator 7.5 705.ipt
- C:\Users\bln15\Documents\GitHub\waffling60\waffling60-XT\Waffling60-MX\Open CASCADE STEP translator 7.5 706.ipt
- C:\Users\bln15\Documents\GitHub\waffling60\waffling60-XT\Waffling60-MX\Open CASCADE STEP translator 7.5 707.ipt
- C:\Users\bln15\Documents\GitHub\waffling60\waffling60-XT\Waffling60-MX\Open CASCADE STEP translator 7.5 708.ipt
- C:\Users\bln15\Documents\GitHub\waffling60\waffling60-XT\Waffling60-MX\Open CASCADE STEP translator 7.5 709.ipt
- C:\Users\bln15\Documents\GitHub\waffling60\waffling60-XT\Waffling60-MX\Open CASCADE STEP translator 7.5 710.ipt
- C:\Users\bln15\Documents\GitHub\waffling60\waffling60-XT\Waffling60-MX\Open CASCADE STEP translator 7.5 711.ipt
- C:\Users\bln15\Documents\GitHub\waffling60\waffling60-XT\Waffling60-MX\Open CASCADE STEP translator 7.5 712.ipt
- C:\Users\bln15\Documents\GitHub\waffling60\waffling60-XT\Waffling60-MX\Open CASCADE STEP translator 7.5 713.ipt
- C:\Users\bln15\Documents\GitHub\waffling60\waffling60-XT\Waffling60-MX\Open CASCADE STEP translator 7.5 714.ipt
- C:\Users\bln15\Documents\GitHub\waffling60\waffling60-XT\Waffling60-MX\Open CASCADE STEP translator 7.5 715.ipt
- C:\Users\bln15\Documents\GitHub\waffling60\waffling60-XT\Waffling60-MX\Open CASCADE STEP translator 7.5 716.ipt
- C:\Users\bln15\Documents\GitHub\waffling60\waffling60-XT\Waffling60-MX\Open CASCADE STEP translator 7.5 717.ipt
- C:\Users\bln15\Documents\GitHub\waffling60\waffling60-XT\Waffling60-MX\Open CASCADE STEP translator 7.5 718.ipt
- C:\Users\bln15\Documents\GitHub\waffling60\waffling60-XT\Waffling60-MX\Open CASCADE STEP translator 7.5 719.ipt
- C:\Users\bln15\Documents\GitHub\waffling60\waffling60-XT\Waffling60-MX\Open CASCADE STEP translator 7.5 720.ipt
- C:\Users\bln15\Documents\GitHub\waffling60\waffling60-XT\Waffling60-MX\Open CASCADE STEP translator 7.5 721.ipt
- C:\Users\bln15\Documents\GitHub\waffling60\waffling60-XT\Waffling60-MX\Open CASCADE STEP translator 7.5 722.ipt
- C:\Users\bln15\Documents\GitHub\waffling60\waffling60-XT\Waffling60-MX\Open CASCADE STEP translator 7.5 723.ipt
- C:\Users\bln15\Documents\GitHub\waffling60\waffling60-XT\Waffling60-MX\Open CASCADE STEP translator 7.5 724.ipt
- C:\Users\bln15\Documents\GitHub\waffling60\waffling60-XT\Waffling60-MX\Open CASCADE STEP translator 7.5 725.ipt
- C:\Users\bln15\Documents\GitHub\waffling60\waffling60-XT\Waffling60-MX\Open CASCADE STEP translator 7.5 726.ipt
- C:\Users\bln15\Documents\GitHub\waffling60\waffling60-XT\Waffling60-MX\Open CASCADE STEP translator 7.5 727.ipt
- C:\Users\bln15\Documents\GitHub\waffling60\waffling60-XT\Waffling60-MX\Open CASCADE STEP translator 7.5 728.ipt
- C:\Users\bln15\Documents\GitHub\waffling60\waffling60-XT\Waffling60-MX\Open CASCADE STEP translator 7.5 729.ipt
- C:\Users\bln15\Documents\GitHub\waffling60\waffling60-XT\Waffling60-MX\Open CASCADE STEP translator 7.5 730.ipt
- C:\Users\bln15\Documents\GitHub\waffling60\waffling60-XT\Waffling60-MX\Open CASCADE STEP translator 7.5 731.ipt
- C:\Users\bln15\Documents\GitHub\waffling60\waffling60-XT\Waffling60-MX\Open CASCADE STEP translator 7.5 732.ipt
- C:\Users\bln15\Documents\GitHub\waffling60\waffling60-XT\Waffling60-MX\Open CASCADE STEP translator 7.5 733.ipt
- C:\Users\bln15\Documents\GitHub\waffling60\waffling60-XT\Waffling60-MX\Open CASCADE STEP translator 7.5 734.ipt
- C:\Users\bln15\Documents\GitHub\waffling60\waffling60-XT\Waffling60-MX\Open CASCADE STEP translator 7.5 735.ipt
- C:\Users\bln15\Documents\GitHub\waffling60\waffling60-XT\Waffling60-MX\Open CASCADE STEP translator 7.5 736.ipt
- C:\Users\bln15\Documents\GitHub\waffling60\waffling60-XT\Waffling60-MX\Open CASCADE STEP translator 7.5 737.ipt
- C:\Users\bln15\Documents\GitHub\waffling60\waffling60-XT\Waffling60-MX\Open CASCADE STEP translator 7.5 738.ipt
- C:\Users\bln15\Documents\GitHub\waffling60\waffling60-XT\Waffling60-MX\Open CASCADE STEP translator 7.5 739.ipt
- C:\Users\bln15\Documents\GitHub\waffling60\waffling60-XT\Waffling60-MX\Open CASCADE STEP translator 7.5 740.ipt
- C:\Users\bln15\Documents\GitHub\waffling60\waffling60-XT\Waffling60-MX\Open CASCADE STEP translator 7.5 741.ipt
- C:\Users\bln15\Documents\GitHub\waffling60\waffling60-XT\Waffling60-MX\Open CASCADE STEP translator 7.5 742.ipt
- C:\Users\bln15\Documents\GitHub\waffling60\waffling60-XT\Waffling60-MX\Open CASCADE STEP translator 7.5 743.ipt
- C:\Users\bln15\Documents\GitHub\waffling60\waffling60-XT\Waffling60-MX\Open CASCADE STEP translator 7.5 744.ipt
- C:\Users\bln15\Documents\GitHub\waffling60\waffling60-XT\Waffling60-MX\Open CASCADE STEP translator 7.5 745.ipt
- C:\Users\bln15\Documents\GitHub\waffling60\waffling60-XT\Waffling60-MX\Open CASCADE STEP translator 7.5 746.ipt
- C:\Users\bln15\Documents\GitHub\waffling60\waffling60-XT\Waffling60-MX\Open CASCADE STEP translator 7.5 747.ipt
- C:\Users\bln15\Documents\GitHub\waffling60\waffling60-XT\Waffling60-MX\Open CASCADE STEP translator 7.5 748.ipt
- C:\Users\bln15\Documents\GitHub\waffling60\waffling60-XT\Waffling60-MX\Open CASCADE STEP translator 7.5 749.ipt
- C:\Users\bln15\Documents\GitHub\waffling60\waffling60-XT\Waffling60-MX\Open CASCADE STEP translator 7.5 750.ipt
- C:\Users\bln15\Documents\GitHub\waffling60\waffling60-XT\Waffling60-MX\Open CASCADE STEP translator 7.5 751.ipt
- C:\Users\bln15\Documents\GitHub\waffling60\waffling60-XT\Waffling60-MX\Open CASCADE STEP translator 7.5 752.ipt
- C:\Users\bln15\Documents\GitHub\waffling60\waffling60-XT\Waffling60-MX\Open CASCADE STEP translator 7.5 753.ipt
- C:\Users\bln15\Documents\GitHub\waffling60\waffling60-XT\Waffling60-MX\Open CASCADE STEP translator 7.5 754.ipt
- C:\Users\bln15\Documents\GitHub\waffling60\waffling60-XT\Waffling60-MX\Open CASCADE STEP translator 7.5 755.ipt
- C:\Users\bln15\Documents\GitHub\waffling60\waffling60-XT\Waffling60-MX\Open CASCADE STEP translator 7.5 756.ipt
- C:\Users\bln15\Documents\GitHub\waffling60\waffling60-XT\Waffling60-MX\Open CASCADE STEP translator 7.5 757.ipt
- C:\Users\bln15\Documents\GitHub\waffling60\waffling60-XT\Waffling60-MX\Open CASCADE STEP translator 7.5 758.ipt
- C:\Users\bln15\Documents\GitHub\waffling60\waffling60-XT\Waffling60-MX\Open CASCADE STEP translator 7.5 759.ipt
- C:\Users\bln15\Documents\GitHub\waffling60\waffling60-XT\Waffling60-MX\Open CASCADE STEP translator 7.5 760.ipt
- C:\Users\bln15\Documents\GitHub\waffling60\waffling60-XT\Waffling60-MX\Open CASCADE STEP translator 7.5 761.ipt
- C:\Users\bln15\Documents\GitHub\waffling60\waffling60-XT\Waffling60-MX\Open CASCADE STEP translator 7.5 762.ipt
- C:\Users\bln15\Documents\GitHub\waffling60\waffling60-XT\Waffling60-MX\Open CASCADE STEP translator 7.5 763.ipt
- C:\Users\bln15\Documents\GitHub\waffling60\waffling60-XT\Waffling60-MX\Open CASCADE STEP translator 7.5 764.ipt
- C:\Users\bln15\Documents\GitHub\waffling60\waffling60-XT\Waffling60-MX\Open CASCADE STEP translator 7.5 765.ipt
- C:\Users\bln15\Documents\GitHub\waffling60\waffling60-XT\Waffling60-MX\Open CASCADE STEP translator 7.5 766.ipt
- C:\Users\bln15\Documents\GitHub\waffling60\waffling60-XT\Waffling60-MX\Open CASCADE STEP translator 7.5 767.ipt
- C:\Users\bln15\Documents\GitHub\waffling60\waffling60-XT\Waffling60-MX\Open CASCADE STEP translator 7.5 768.ipt
- C:\Users\bln15\Documents\GitHub\waffling60\waffling60-XT\Waffling60-MX\Open CASCADE STEP translator 7.5 769.ipt
- C:\Users\bln15\Documents\GitHub\waffling60\waffling60-XT\Waffling60-MX\Open CASCADE STEP translator 7.5 770.ipt
- C:\Users\bln15\Documents\GitHub\waffling60\waffling60-XT\Waffling60-MX\Open CASCADE STEP translator 7.5 771.ipt
- C:\Users\bln15\Documents\GitHub\waffling60\waffling60-XT\Waffling60-MX\Open CASCADE STEP translator 7.5 772.ipt
- C:\Users\bln15\Documents\GitHub\waffling60\waffling60-XT\Waffling60-MX\Open CASCADE STEP translator 7.5 773.ipt
- C:\Users\bln15\Documents\GitHub\waffling60\waffling60-XT\Waffling60-MX\Open CASCADE STEP translator 7.5 774.ipt
- C:\Users\bln15\Documents\GitHub\waffling60\waffling60-XT\Waffling60-MX\Open CASCADE STEP translator 7.5 775.ipt
- C:\Users\bln15\Documents\GitHub\waffling60\waffling60-XT\Waffling60-MX\Open CASCADE STEP translator 7.5 776.ipt
- C:\Users\bln15\Documents\GitHub\waffling60\waffling60-XT\Waffling60-MX\Open CASCADE STEP translator 7.5 777.ipt
- C:\Users\bln15\Documents\GitHub\waffling60\waffling60-XT\Waffling60-MX\Open CASCADE STEP translator 7.5 778.ipt
- C:\Users\bln15\Documents\GitHub\waffling60\waffling60-XT\Waffling60-MX\Open CASCADE STEP translator 7.5 779.ipt
- C:\Users\bln15\Documents\GitHub\waffling60\waffling60-XT\Waffling60-MX\Open CASCADE STEP translator 7.5 780.ipt
- C:\Users\bln15\Documents\GitHub\waffling60\waffling60-XT\Waffling60-MX\Open CASCADE STEP translator 7.5 781.ipt
- C:\Users\bln15\Documents\GitHub\waffling60\waffling60-XT\Waffling60-MX\Open CASCADE STEP translator 7.5 782.ipt
- C:\Users\bln15\Documents\GitHub\waffling60\waffling60-XT\Waffling60-MX\Open CASCADE STEP translator 7.5 783.ipt
- C:\Users\bln15\Documents\GitHub\waffling60\waffling60-XT\Waffling60-MX\Open CASCADE STEP translator 7.5 784.ipt
- C:\Users\bln15\Documents\GitHub\waffling60\waffling60-XT\Waffling60-MX\Open CASCADE STEP translator 7.5 785.ipt
- C:\Users\bln15\Documents\GitHub\waffling60\waffling60-XT\Waffling60-MX\Open CASCADE STEP translator 7.5 786.ipt
- C:\Users\bln15\Documents\GitHub\waffling60\waffling60-XT\Waffling60-MX\Open CASCADE STEP translator 7.5 787.ipt
- C:\Users\bln15\Documents\GitHub\waffling60\waffling60-XT\Waffling60-MX\Open CASCADE STEP translator 7.5 788.ipt
- C:\Users\bln15\Documents\GitHub\waffling60\waffling60-XT\Waffling60-MX\Open CASCADE STEP translator 7.5 789.ipt
- C:\Users\bln15\Documents\GitHub\waffling60\waffling60-XT\Waffling60-MX\Open CASCADE STEP translator 7.5 790.ipt
- C:\Users\bln15\Documents\GitHub\waffling60\waffling60-XT\Waffling60-MX\Open CASCADE STEP translator 7.5 791.ipt
- C:\Users\bln15\Documents\GitHub\waffling60\waffling60-XT\Waffling60-MX\Open CASCADE STEP translator 7.5 792.ipt
- C:\Users\bln15\Documents\GitHub\waffling60\waffling60-XT\Waffling60-MX\Open CASCADE STEP translator 7.5 793.ipt
- C:\Users\bln15\Documents\GitHub\waffling60\waffling60-XT\Waffling60-MX\Open CASCADE STEP translator 7.5 794.ipt
- C:\Users\bln15\Documents\GitHub\waffling60\waffling60-XT\Waffling60-MX\Open CASCADE STEP translator 7.5 795.ipt
- C:\Users\bln15\Documents\GitHub\waffling60\waffling60-XT\Waffling60-MX\Open CASCADE STEP translator 7.5 796.ipt
- C:\Users\bln15\Documents\GitHub\waffling60\waffling60-XT\Waffling60-MX\Open CASCADE STEP translator 7.5 797.ipt
- C:\Users\bln15\Documents\GitHub\waffling60\waffling60-XT\Waffling60-MX\Open CASCADE STEP translator 7.5 798.ipt
- C:\Users\bln15\Documents\GitHub\waffling60\waffling60-XT\Waffling60-MX\Open CASCADE STEP translator 7.5 799.ipt
- C:\Users\bln15\Documents\GitHub\waffling60\waffling60-XT\Waffling60-MX\Open CASCADE STEP translator 7.5 800.ipt
- C:\Users\bln15\Documents\GitHub\waffling60\waffling60-XT\Waffling60-MX\Open CASCADE STEP translator 7.5 801.ipt
- C:\Users\bln15\Documents\GitHub\waffling60\waffling60-XT\Waffling60-MX\Open CASCADE STEP translator 7.5 802.ipt
- C:\Users\bln15\Documents\GitHub\waffling60\waffling60-XT\Waffling60-MX\Open CASCADE STEP translator 7.5 803.ipt
- C:\Users\bln15\Documents\GitHub\waffling60\waffling60-XT\Waffling60-MX\Open CASCADE STEP translator 7.5 804.ipt
- C:\Users\bln15\Documents\GitHub\waffling60\waffling60-XT\Waffling60-MX\Open CASCADE STEP translator 7.5 805.ipt
- C:\Users\bln15\Documents\GitHub\waffling60\waffling60-XT\Waffling60-MX\Open CASCADE STEP translator 7.5 806.ipt
- C:\Users\bln15\Documents\GitHub\waffling60\waffling60-XT\Waffling60-MX\Open CASCADE STEP translator 7.5 807.ipt
- C:\Users\bln15\Documents\GitHub\waffling60\waffling60-XT\Waffling60-MX\Open CASCADE STEP translator 7.5 808.ipt
- C:\Users\bln15\Documents\GitHub\waffling60\waffling60-XT\Waffling60-MX\Open CASCADE STEP translator 7.5 809.ipt
- C:\Users\bln15\Documents\GitHub\waffling60\waffling60-XT\Waffling60-MX\Open CASCADE STEP translator 7.5 810.ipt
- C:\Users\bln15\Documents\GitHub\waffling60\waffling60-XT\Waffling60-MX\Open CASCADE STEP translator 7.5 811.ipt
- C:\Users\bln15\Documents\GitHub\waffling60\waffling60-XT\Waffling60-MX\Open CASCADE STEP translator 7.5 812.ipt
- C:\Users\bln15\Documents\GitHub\waffling60\waffling60-XT\Waffling60-MX\Open CASCADE STEP translator 7.5 813.ipt
- C:\Users\bln15\Documents\GitHub\waffling60\waffling60-XT\Waffling60-MX\Open CASCADE STEP translator 7.5 814.ipt
- C:\Users\bln15\Documents\GitHub\waffling60\waffling60-XT\Waffling60-MX\Open CASCADE STEP translator 7.5 815.ipt
- C:\Users\bln15\Documents\GitHub\waffling60\waffling60-XT\Waffling60-MX\Open CASCADE STEP translator 7.5 816.ipt
- C:\Users\bln15\Documents\GitHub\waffling60\waffling60-XT\Waffling60-MX\Open CASCADE STEP translator 7.5 817.ipt
- C:\Users\bln15\Documents\GitHub\waffling60\waffling60-XT\Waffling60-MX\Open CASCADE STEP translator 7.5 818.ipt
- C:\Users\bln15\Documents\GitHub\waffling60\waffling60-XT\Waffling60-MX\Open CASCADE STEP translator 7.5 819.ipt
- C:\Users\bln15\Documents\GitHub\waffling60\waffling60-XT\Waffling60-MX\Open CASCADE STEP translator 7.5 820.ipt
- C:\Users\bln15\Documents\GitHub\waffling60\waffling60-XT\Waffling60-MX\Open CASCADE STEP translator 7.5 821.ipt
- C:\Users\bln15\Documents\GitHub\waffling60\waffling60-XT\Waffling60-MX\Open CASCADE STEP translator 7.5 822.ipt
- C:\Users\bln15\Documents\GitHub\waffling60\waffling60-XT\Waffling60-MX\Open CASCADE STEP translator 7.5 823.ipt
- C:\Users\bln15\Documents\GitHub\waffling60\waffling60-XT\Waffling60-MX\Open CASCADE STEP translator 7.5 824.ipt
## Components (412 placed, 412 different names)
1. Open CASCADE STEP translator 7.5 413
2. Open CASCADE STEP translator 7.5 414
3. Open CASCADE STEP translator 7.5 415
4. Open CASCADE STEP translator 7.5 416
5. Open CASCADE STEP translator 7.5 417
6. Open CASCADE STEP translator 7.5 418
7. Open CASCADE STEP translator 7.5 419
8. Open CASCADE STEP translator 7.5 420
9. Open CASCADE STEP translator 7.5 421
10. Open CASCADE STEP translator 7.5 422
11. Open CASCADE STEP translator 7.5 423
12. Open CASCADE STEP translator 7.5 424
13. Open CASCADE STEP translator 7.5 425
14. Open CASCADE STEP translator 7.5 426
15. Open CASCADE STEP translator 7.5 427
16. Open CASCADE STEP translator 7.5 428
17. Open CASCADE STEP translator 7.5 429
18. Open CASCADE STEP translator 7.5 430
19. Open CASCADE STEP translator 7.5 431
20. Open CASCADE STEP translator 7.5 432
21. Open CASCADE STEP translator 7.5 433
22. Open CASCADE STEP translator 7.5 434
23. Open CASCADE STEP translator 7.5 435
24. Open CASCADE STEP translator 7.5 436
25. Open CASCADE STEP translator 7.5 437
26. Open CASCADE STEP translator 7.5 438
27. Open CASCADE STEP translator 7.5 439
28. Open CASCADE STEP translator 7.5 440
29. Open CASCADE STEP translator 7.5 441
30. Open CASCADE STEP translator 7.5 442
31. Open CASCADE STEP translator 7.5 443
32. Open CASCADE STEP translator 7.5 444
33. Open CASCADE STEP translator 7.5 445
34. Open CASCADE STEP translator 7.5 446
35. Open CASCADE STEP translator 7.5 447
36. Open CASCADE STEP translator 7.5 448
37. Open CASCADE STEP translator 7.5 449
38. Open CASCADE STEP translator 7.5 450
39. Open CASCADE STEP translator 7.5 451
40. Open CASCADE STEP translator 7.5 452
41. Open CASCADE STEP translator 7.5 453
42. Open CASCADE STEP translator 7.5 454
43. Open CASCADE STEP translator 7.5 455
44. Open CASCADE STEP translator 7.5 456
45. Open CASCADE STEP translator 7.5 457
46. Open CASCADE STEP translator 7.5 458
47. Open CASCADE STEP translator 7.5 459
48. Open CASCADE STEP translator 7.5 460
49. Open CASCADE STEP translator 7.5 461
50. Open CASCADE STEP translator 7.5 462
51. Open CASCADE STEP translator 7.5 463
52. Open CASCADE STEP translator 7.5 464
53. Open CASCADE STEP translator 7.5 465
54. Open CASCADE STEP translator 7.5 466
55. Open CASCADE STEP translator 7.5 467